# Autodesk Inventor assembly: Cremallera
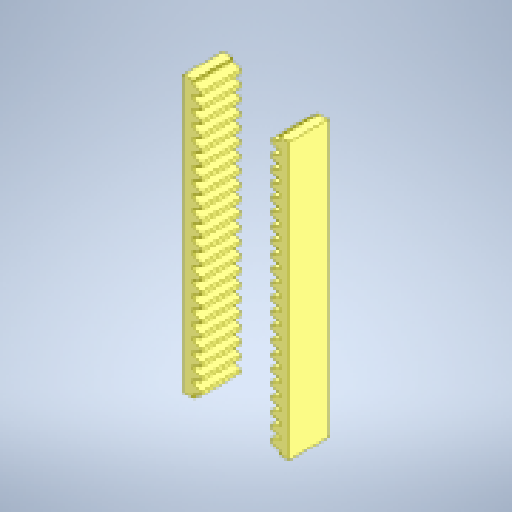
[picture p0: Inventor's stored thumbnail of the model, 512x512]
Saved by Autodesk Inventor 2024 (Build 280153000, 153)
## iProperties
Created: 2025-03-04
Part Number: Cremallera
Document SubType Name: Assembly
Designer: sergi
Author: sergi
## Documents named in this file (5)
- C:\Users\sergi\OneDrive\Escritorio\Projects\16. Protection catapult\Inventor\Cremallera.iam
- C:\Users\sergi\OneDrive\Escritorio\Projects\16. Protection catapult\Inventor\Tope.ipt
- C:\Users\sergi\OneDrive\Escritorio\Projects\16. Protection catapult\Inventor\Tope trasero.ipt
- C:\Users\sergi\OneDrive\Escritorio\Projects\16. Protection catapult\Inventor\103005_para_cremalleras_1\103005_para_cremalleras_1.ipt
- C:\Users\sergi\OneDrive\Escritorio\Projects\16. Protection catapult\Inventor\Tirante.ipt
## Components (5 placed, 4 different names)
1. Tope:1 — Nivelación:1, Nivelación:2, Coincidencia:1, Coincidencia:2, Nivelación:3, Nivelación:4, Nivelación:7, Nivelación:8
2. Tope trasero:1 — Coincidencia:3, Nivelación:5, Nivelación:6
3. 103005_para_cremalleras_1:1 — Coincidencia:2, Nivelación:3, Nivelación:4
4. 103005_para_cremalleras_1:2 — Nivelación:1, Nivelación:2, Coincidencia:1, Coincidencia:3, Nivelación:5, Nivelación:6
5. Tirante:1 — Nivelación:7, Nivelación:8
## Relationships (11: Flush 8, Mate 3)
- Nivelación:1 [Flush]: Tope:1 ↔ 103005_para_cremalleras_1:2
- Nivelación:2 [Flush]: Tope:1 ↔ 103005_para_cremalleras_1:2
- Coincidencia:1 [Mate]: Tope:1 ↔ 103005_para_cremalleras_1:2
- Coincidencia:2 [Mate]: Tope:1 ↔ 103005_para_cremalleras_1:1
- Nivelación:3 [Flush]: Tope:1 ↔ 103005_para_cremalleras_1:1
- Nivelación:4 [Flush]: Tope:1 ↔ 103005_para_cremalleras_1:1
- Coincidencia:3 [Mate]: Tope trasero:1 ↔ 103005_para_cremalleras_1:2
- Nivelación:5 [Flush]: Tope trasero:1 ↔ 103005_para_cremalleras_1:2
- Nivelación:6 [Flush]: Tope trasero:1 ↔ 103005_para_cremalleras_1:2
- Nivelación:7 [Flush]: Tope:1 ↔ Tirante:1
- Nivelación:8 [Flush]: Tope:1 ↔ Tirante:1
